# Autodesk Inventor assembly: TAKE UP UNIT
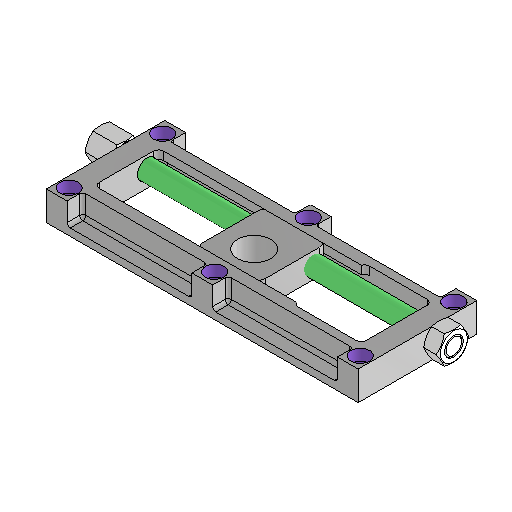
[picture p0: Inventor's stored thumbnail of the model, 512x512]
Saved by Autodesk Inventor 2022.5 (Build 265521000, 521)
## iProperties
RuleStatus: InUse
Created: 2024-07-18
Part Number: TAKE UP UNIT
Material: SS400
Description: 3
Document SubType Name: Assembly
Designer: USER106
MAKER: SHINWOO
Deteil Description: Detail Description
Detail Description: Purchased products
Title: CTSN-9
Author: USER106
Revision Number: A
## Documents named in this file (4)
- D:\V\Designs\구매품(업체별)\기타\TAKE UP UNIT_CTSN-9_SHINWOO.iam
- D:\V\Designs\구매품(업체별)\기타\TAKE UP UNIT_CTSN-9(BODY)_SHINWOO.ipt
- D:\V\Designs\구매품(업체별)\기타\TAKE UP UNIT_CTSN-9(ROD)_SHINWOO.ipt
- D:\V\Designs\구매품(업체별)\기타\TAKE UP UNIT_CTSN-9(PISTON)_SHINWOO.ipt
## Components (3 placed, 3 different names)
1. TAKE UP UNIT_CTSN-9(BODY)_SHINWOO.ipt:1 — Mate:1, Mate:3, Mate:4, Angle:1, ORIGIN, Mate:8
2. TAKE UP UNIT_CTSN-9(PISTON)_SHINWOO.ipt:1 — Mate:2, Mate:3, ORIGIN, Mate:8
3. TAKE UP UNIT_CTSN-9(ROD)_SHINWOO.ipt:1 — Mate:1, Mate:2, Mate:4, Angle:1
## Relationships (7: Mate 6, Angle 1)
- Mate:1: TAKE UP UNIT_CTSN-9(BODY)_SHINWOO.ipt:1 ↔ TAKE UP UNIT_CTSN-9(ROD)_SHINWOO.ipt:1
- Mate:2: TAKE UP UNIT_CTSN-9(PISTON)_SHINWOO.ipt:1 ↔ TAKE UP UNIT_CTSN-9(ROD)_SHINWOO.ipt:1
- Mate:3: TAKE UP UNIT_CTSN-9(BODY)_SHINWOO.ipt:1 ↔ TAKE UP UNIT_CTSN-9(PISTON)_SHINWOO.ipt:1
- Mate:4: TAKE UP UNIT_CTSN-9(BODY)_SHINWOO.ipt:1 ↔ TAKE UP UNIT_CTSN-9(ROD)_SHINWOO.ipt:1
- Angle:1 (0 deg): TAKE UP UNIT_CTSN-9(BODY)_SHINWOO.ipt:1 ↔ TAKE UP UNIT_CTSN-9(ROD)_SHINWOO.ipt:1
- ORIGIN [Mate] (100 mm): TAKE UP UNIT_CTSN-9(BODY)_SHINWOO.ipt:1 ↔ TAKE UP UNIT_CTSN-9(PISTON)_SHINWOO.ipt:1
- Mate:8: TAKE UP UNIT_CTSN-9(BODY)_SHINWOO.ipt:1 ↔ TAKE UP UNIT_CTSN-9(PISTON)_SHINWOO.ipt:1
